# Autodesk Inventor assembly: Tower
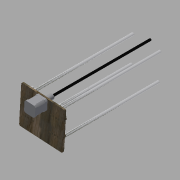
[picture p0: Inventor's stored thumbnail of the model, 180x180]
Saved by Autodesk Inventor 2019 (Build 230136000, 136)
## iProperties
Created: 2021-11-03
Part Number: Tower
Document SubType Name: Assembly
Designer: Mohamed
Author: Mohamed
## Documents named in this file (8)
- F:\Semester 7\Design of mechatronics 1\SSCARA Robot\Tower.iam
- F:\Semester 7\Design of mechatronics 1\SSCARA Robot\e_lead.ipt
- F:\Semester 7\Design of mechatronics 1\SSCARA Robot\e_coupler.ipt
- F:\Semester 7\Design of mechatronics 1\SSCARA Robot\e_circuler rod 400mm.ipt
- F:\Semester 7\Design of mechatronics 1\SSCARA Robot\e_top 1.ipt
- F:\Semester 7\Design of mechatronics 1\SSCARA Robot\e_linear rail support.ipt
- F:\Semester 7\Design of mechatronics 1\SSCARA Robot\nema 17 motor.ipt
- F:\Semester 7\Design of mechatronics 1\SSCARA Robot\e_rail support.ipt
## Components (16 placed, 7 different names)
1. e_top 1:1 — Mate:5, Mate:6, Mate:7, Mate:8, Mate:11, Mate:12, Mate:13, Flush:3, Flush:4, Flush:5, Flush:6, Mate:22, Mate:23, Mate:24, Mate:25, Mate:26, Mate:27, Mate:29, Mate:33, Mate:34, Mate:35
2. e_linear rail support:1 — Mate:5, Flush:1, Mate:14, Mate:19, Mate:30
3. e_linear rail support:2 — Mate:8, Flush:1, Mate:15, Mate:18, Mate:31
4. e_linear rail support:3 — Mate:7, Flush:2, Mate:17, Mate:21, Mate:32
5. e_linear rail support:4 — Mate:6, Flush:2, Mate:16, Mate:20, Mate:28
6. nema 17 motor:1 — Mate:11, Mate:12, Mate:13, Mate:38, Mate:39
7. e_rail support:1 — Flush:3, Mate:14, Mate:19, Mate:26, Mate:27
8. e_rail support:2 — Flush:4, Mate:15, Mate:18, Mate:25
9. e_rail support:3 — Flush:5, Mate:16, Mate:20, Mate:22, Mate:23
10. e_rail support:4 — Flush:6, Mate:17, Mate:21, Mate:24
11. e_circuler rod 400mm:1 — Mate:30, Mate:34
12. e_circuler rod 400mm:2 — Mate:31, Mate:33
13. e_circuler rod 400mm:3 — Mate:32, Mate:35
14. e_circuler rod 400mm:4 — Mate:28, Mate:29
15. e_coupler:1 — Mate:36, Mate:37, Mate:38
16. e_lead:1 — Mate:36, Mate:37, Mate:39
## Relationships (39: Mate 33, Flush 6)
- Mate:5: e_top 1:1 ↔ e_linear rail support:1
- Mate:6: e_top 1:1 ↔ e_linear rail support:4
- Mate:7: e_top 1:1 ↔ e_linear rail support:3
- Mate:8: e_top 1:1 ↔ e_linear rail support:2
- Flush:1: e_linear rail support:1 ↔ e_linear rail support:2
- Flush:2: e_linear rail support:3 ↔ e_linear rail support:4
- Mate:11: e_top 1:1 ↔ nema 17 motor:1
- Mate:12: e_top 1:1 ↔ nema 17 motor:1
- Mate:13: e_top 1:1 ↔ nema 17 motor:1
- Flush:3: e_top 1:1 ↔ e_rail support:1
- Flush:4: e_top 1:1 ↔ e_rail support:2
- Flush:5: e_top 1:1 ↔ e_rail support:3
- Flush:6: e_top 1:1 ↔ e_rail support:4
- Mate:14: e_linear rail support:1 ↔ e_rail support:1
- Mate:15: e_linear rail support:2 ↔ e_rail support:2
- Mate:16: e_linear rail support:4 ↔ e_rail support:3
- Mate:17: e_linear rail support:3 ↔ e_rail support:4
- Mate:18: e_linear rail support:2 ↔ e_rail support:2
- Mate:19: e_linear rail support:1 ↔ e_rail support:1
- Mate:20: e_linear rail support:4 ↔ e_rail support:3
- Mate:21: e_linear rail support:3 ↔ e_rail support:4
- Mate:22: e_top 1:1 ↔ e_rail support:3
- Mate:23: e_top 1:1 ↔ e_rail support:3
- Mate:24: e_top 1:1 ↔ e_rail support:4
- Mate:25: e_top 1:1 ↔ e_rail support:2
- Mate:26: e_top 1:1 ↔ e_rail support:1
- Mate:27: e_top 1:1 ↔ e_rail support:1
- Mate:28: e_linear rail support:4 ↔ e_circuler rod 400mm:4
- Mate:29: e_top 1:1 ↔ e_circuler rod 400mm:4
- Mate:30: e_linear rail support:1 ↔ e_circuler rod 400mm:1
- Mate:31: e_linear rail support:2 ↔ e_circuler rod 400mm:2
- Mate:32: e_linear rail support:3 ↔ e_circuler rod 400mm:3
- Mate:33: e_top 1:1 ↔ e_circuler rod 400mm:2
- Mate:34: e_top 1:1 ↔ e_circuler rod 400mm:1
- Mate:35: e_top 1:1 ↔ e_circuler rod 400mm:3
- Mate:36: e_coupler:1 ↔ e_lead:1
- Mate:37: e_coupler:1 ↔ e_lead:1
- Mate:38: nema 17 motor:1 ↔ e_coupler:1
- Mate:39: nema 17 motor:1 ↔ e_lead:1
